# Autodesk Inventor assembly: 11527¹à·â¹¤³ÌÍ¼
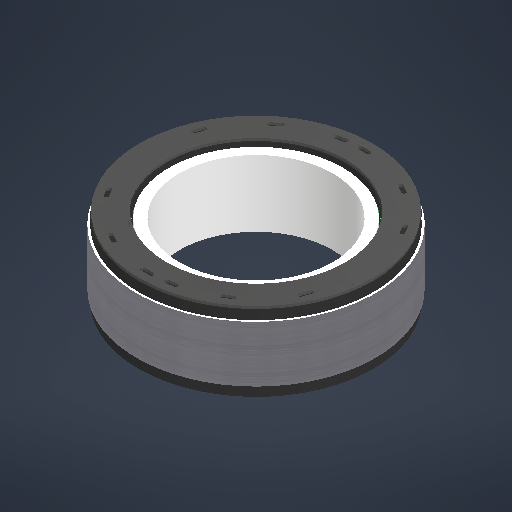
[picture p0: Inventor's stored thumbnail of the model, 512x512]
Saved by Autodesk Inventor 2026.1 (Build 301233000, 233)
## iProperties
Created: 2023-12-21
Part Number: 11527¹à·â¹¤³ÌÍ¼
Description: STEP AP214
Document SubType Name: Assembly
Designer: aaron
Sending System: SolidWorks 2020
Preprocessor: SwSTEP 2.0
Title: 11527¹à·â¹¤³ÌÍ¼.STEP
Author: tmotor
Revision Number: ÈÎºÎ
## Documents named in this file (4)
- D:\work\loopandpixel\openworkoutsystem\cad\v5\RI115-PH\RI115-PH.iam
- D:\work\loopandpixel\openworkoutsystem\cad\v5\RI115-PH\11527ÌúÐ¾-¹à·â.ipt
- D:\work\loopandpixel\openworkoutsystem\cad\v5\RI115-PH\115 PCB-¹¤³ÌÍ¼ÓÃ.ipt
- D:\work\loopandpixel\openworkoutsystem\cad\v5\RI115-PH\11527×ª×Ó-¼Ó³¤.iam
## Components (3 placed, 3 different names)
1. 11527ÌúÐ¾-¹à·â_1 — Insert:1
2. 115 PCB-¹¤³ÌÍ¼ÓÃ_2
3. 11527×ª×Ó-¼Ó³¤_3 [sub-assembly] — Insert:1
## Relationships (1: Insert 1)
- Insert:1 (2.8 mm): 11527ÌúÐ¾-¹à·â_1 ↔ 11527×ª×Ó-¼Ó³¤_3
